# Autodesk Inventor assembly: WheelIntake5.0Mirror
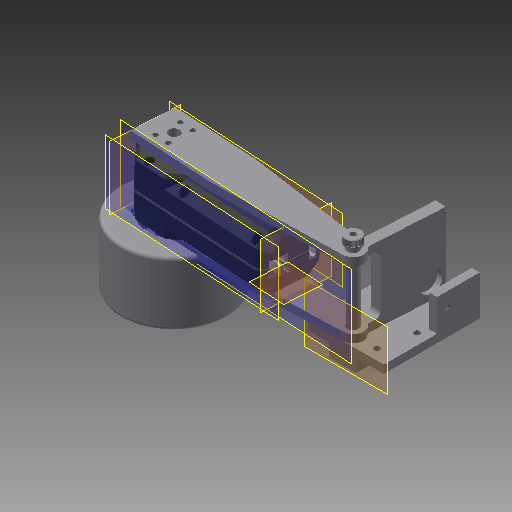
[picture p0: Inventor's stored thumbnail of the model, 512x512]
Saved by Autodesk Inventor 2017 (Build 210142000, 142)
## iProperties
Created: 2017-12-16
Part Number: WheelIntake5.0Mirror
Document SubType Name: Assembly
Designer: User
Author: User
## Documents named in this file (6)
- C:\Robotics\CAD\2017-18_CAD\WheelIntake5.0Mirror.iam
- C:\Robotics\CAD\2017-18_CAD\WheelIntake5.0MountMirror.ipt
- C:\Robotics\CAD\2017-18_CAD\WheelIntake5.0BaseMirror.ipt
- C:\Robotics\CAD\COTSParts\Rev\REV-41-1300HexMotor.ipt
- C:\Robotics\CAD\COTSParts\Fasteners\97345A171_TYPE 316 STAINLESS STEEL SHOULDER SCREW.ipt
- C:\Robotics\CAD\COTSParts\Wheels\2.5inFoamWheel250TMD.ipt
## Components (5 placed, 5 different names)
1. WheelIntake5.0MountMirror:1 — Insert:2, Insert:3, Insert:4, Insert:5
2. WheelIntake5.0BaseMirror:1 — Insert:1
3. REV-41-1300HexMotor:1 — Insert:3, Insert:4
4. 97345A171_TYPE 316 STAINLESS STEEL SHOULDER SCREW:1 — Insert:1, Insert:2
5. 2.5inFoamWheel250TMD:1 — Insert:5
## Relationships (5: Insert 5)
- Insert:1: WheelIntake5.0BaseMirror:1 ↔ 97345A171_TYPE 316 STAINLESS STEEL SHOULDER SCREW:1
- Insert:2: WheelIntake5.0MountMirror:1 ↔ 97345A171_TYPE 316 STAINLESS STEEL SHOULDER SCREW:1
- Insert:3: WheelIntake5.0MountMirror:1 ↔ REV-41-1300HexMotor:1
- Insert:4: WheelIntake5.0MountMirror:1 ↔ REV-41-1300HexMotor:1
- Insert:5: WheelIntake5.0MountMirror:1 ↔ 2.5inFoamWheel250TMD:1
